# Autodesk Inventor assembly: cylinderAssembly
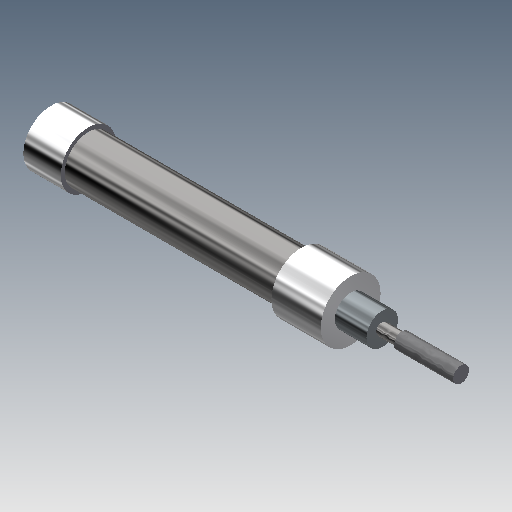
[picture p0: Inventor's stored thumbnail of the model, 512x512]
Saved by Autodesk Inventor 2017 (Build 210142000, 142)
## iProperties
Created: 2018-05-01
Part Number: cylinderAssembly
Document SubType Name: Assembly
Designer: Luiz Gustavo
Author: Luiz Gustavo
## Documents named in this file (3)
- C:\Users\Luiz Gustavo\Documents\Inventor\piano-robot\cylinderAssembly.iam
- C:\Users\Luiz Gustavo\Documents\Inventor\piano-robot\30mmCylinder.ipt
- C:\Users\Luiz Gustavo\Documents\Inventor\piano-robot\cylinderRod.ipt
## Components (2 placed, 2 different names)
1. 30mmCylinder:1 — Flush:2, Flush:3, Flush:4, Flush:5
2. cylinderRod:1 — Flush:5, Flush:6, Mate:1
## Relationships (6: Flush 5, Mate 1)
- Flush:2: 30mmCylinder:1
- Flush:3: 30mmCylinder:1
- Flush:4: 30mmCylinder:1
- Flush:5 (28 mm): 30mmCylinder:1 ↔ cylinderRod:1
- Flush:6: cylinderRod:1
- Mate:1: cylinderRod:1
## Named parameters: parA = 15 mm, parB = 12 mm, parC = 14 mm, parD = 4 mm, parF = 8 mm, parGA = 8 mm, parGB = 5 mm, parH = 28 mm, parMM = 4 mm, parNA = 12.5 mm, parNB = 9.5 mm, Ndh8 = 8 mm, parNN = 8 mm, parS = 46 mm, parZ = 74 mm, stroke = 30 mm
